# Autodesk Inventor assembly: Assembly1
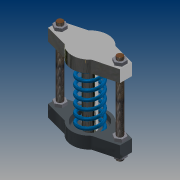
[picture p0: Inventor's stored thumbnail of the model, 180x180]
Saved by Autodesk Inventor 2014 (Build 180170000, 170)
## iProperties
Created: 2021-03-21
Part Number: Assembly1
Document SubType Name: Assembly
Designer: Think Station
Mass: 1181.85 g
Surface Area: 692.71 cm^2
Volume: 219.874 cm^3
Density: 5.37516 g/cm^3
Author: Think Station
## Documents named in this file (6)
- E:\Entraco_Diptanshu\3D\##TEST##\Spring Simulation\Assembly1.iam
- E:\Entraco_Diptanshu\3D\##TEST##\Spring Simulation\BOTTOM.ipt
- E:\Entraco_Diptanshu\3D\##TEST##\Spring Simulation\TOP.ipt
- E:\Entraco_Diptanshu\3D\##TEST##\Spring Simulation\SPRING.ipt
- E:\Entraco_Diptanshu\3D\##TEST##\Spring Simulation\BOLT.ipt
- C:\Users\Think Station\Documents\Inventor\Content Center Files\R2014\en-US\DIN EN 24 036(2)\DIN EN 24 036 - M10.ipt
## Components (11 placed, 5 different names)
1. BOTTOM:1 — Mate:1, Flush:1, Mate:5, Mate:6, Flush:2, Mate:8, Flush:3, Mate:10, Mate:12, Mate:18, Mate:20
2. TOP:1 — Mate:1, Flush:1, Mate:3, Mate:4, Mate:6, Mate:7, Mate:15, Mate:16
3. SPRING:1 — Mate:3, Mate:4, Mate:5
4. BOLT:1 — Mate:7, Flush:2, Mate:11, Mate:14, Mate:17
5. BOLT:2 — Mate:8, Flush:3, Mate:9, Mate:13, Mate:19
6. DIN EN 24036 M10:1 — Mate:9, Mate:10
7. DIN EN 24036 M10:2 — Mate:11, Mate:12
8. DIN EN 24036 M10:3 — Mate:13, Mate:16
9. DIN EN 24036 M10:4 — Mate:14, Mate:15
10. DIN EN 24036 M10:5 — Mate:17, Mate:18
11. DIN EN 24036 M10:6 — Mate:19, Mate:20
## Relationships (22: Mate 19, Flush 3)
- Mate:1: BOTTOM:1 ↔ TOP:1
- Flush:1: BOTTOM:1 ↔ TOP:1
- Mate:3: TOP:1 ↔ SPRING:1
- Mate:4: TOP:1 ↔ SPRING:1
- Mate:5: BOTTOM:1 ↔ SPRING:1
- Mate:6 (90 mm): BOTTOM:1 ↔ TOP:1
- Mate:7: TOP:1 ↔ BOLT:1
- Flush:2 (-10 mm): BOTTOM:1 ↔ BOLT:1
- Mate:8: BOTTOM:1 ↔ BOLT:2
- Flush:3 (10 mm): BOTTOM:1 ↔ BOLT:2
- Mate:9: BOLT:2 ↔ DIN EN 24036 M10:1
- Mate:10: BOTTOM:1 ↔ DIN EN 24036 M10:1
- Mate:11: BOLT:1 ↔ DIN EN 24036 M10:2
- Mate:12: BOTTOM:1 ↔ DIN EN 24036 M10:2
- Mate:13: BOLT:2 ↔ DIN EN 24036 M10:3
- Mate:14: BOLT:1 ↔ DIN EN 24036 M10:4
- Mate:15: TOP:1 ↔ DIN EN 24036 M10:4
- Mate:16: TOP:1 ↔ DIN EN 24036 M10:3
- Mate:17: BOLT:1 ↔ DIN EN 24036 M10:5
- Mate:18: BOTTOM:1 ↔ DIN EN 24036 M10:5
- Mate:19: BOLT:2 ↔ DIN EN 24036 M10:6
- Mate:20: BOTTOM:1 ↔ DIN EN 24036 M10:6
